# Autodesk Inventor assembly: 基本構造距離センサ2セット配置
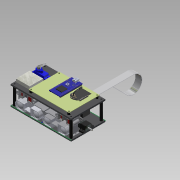
[picture p0: Inventor's stored thumbnail of the model, 180x180]
Saved by Autodesk Inventor 2017 (Build 210142000, 142)
## iProperties
Part Number: 基本構造距離センサ2セット配置
Material: 一般
Document SubType Name: Assembly
Designer: HISAAKI
Author: HISAAKI
## Documents named in this file (19)
- C:\Users\HISAAKI\Documents\LYNCS\CanSat\2017種子島\cansat-structure\基本構造距離センサ2セット配置.iam
- C:\Users\HISAAKI\Documents\LYNCS\CanSat\2017種子島\cansat-structure\既成部品\ブラケット.ipt
- C:\Users\HISAAKI\Documents\LYNCS\CanSat\2017種子島\cansat-structure\既成部品\モータ.ipt
- C:\Users\HISAAKI\Documents\LYNCS\CanSat\2017種子島\cansat-structure\ハブver1.1.ipt
- C:\Users\HISAAKI\Documents\LYNCS\CanSat\2017種子島\cansat-structure\タイヤスポンジ部分.ipt
- C:\Users\HISAAKI\Documents\LYNCS\CanSat\2017種子島\cansat-structure\基本板上.ipt
- C:\Users\HISAAKI\Documents\LYNCS\CanSat\2017種子島\cansat-structure\既成部品\スペーサ.ipt
- C:\Users\HISAAKI\Documents\LYNCS\CanSat\2017種子島\cansat-structure\既成部品\GPSユニット.ipt
- C:\Users\HISAAKI\Documents\LYNCS\CanSat\2017種子島\cansat-structure\基板.ipt
- C:\Users\HISAAKI\Documents\LYNCS\CanSat\2017種子島\cansat-structure\スペーサ5mm.ipt
- C:\Users\HISAAKI\Documents\LYNCS\CanSat\2017種子島\cansat-structure\タイヤプラ板部分.ipt
- C:\Users\HISAAKI\Documents\LYNCS\CanSat\2017種子島\cansat-structure\スタビライザ.ipt
- C:\Users\HISAAKI\Documents\LYNCS\CanSat\2017種子島\cansat-structure\リポ電池黒.ipt
- C:\Users\HISAAKI\Documents\LYNCS\CanSat\2017種子島\cansat-structure\mbed_NXP_LPC1768.ipt
- C:\Users\HISAAKI\Documents\LYNCS\CanSat\2017種子島\cansat-structure\センサ2個積み右.iam
- C:\Users\HISAAKI\Documents\LYNCS\CanSat\2017種子島\cansat-structure\センサ2セット積み左.iam
- C:\Users\HISAAKI\Documents\LYNCS\CanSat\2017種子島\cansat-structure\XBeeProS1.ipt
- C:\Users\HISAAKI\Documents\LYNCS\CanSat\2017種子島\cansat-structure\Tower Pro 9g Micro Servo SG90.ipt
- C:\Users\HISAAKI\Documents\LYNCS\CanSat\2017種子島\cansat-structure\基本板().ipt
## Components (30 placed, 18 different names)
1. モータ:1 — メイト:13, メイト:14, メイト:41, メイト:43, フラッシュ:106
2. モータ:2 — メイト:11, メイト:12, メイト:42, メイト:44, フラッシュ:105
3. ハブver1.1:1 — メイト:11, メイト:12, メイト:17, メイト:18
4. ハブver1.1:2 — メイト:13, メイト:14, メイト:15, メイト:16
5. タイヤスポンジ部分:1 — メイト:15, メイト:16, メイト:62, メイト:63
6. タイヤスポンジ部分:2 — メイト:17, メイト:18, メイト:64, メイト:65
7. 基本板上:1 — メイト:31, メイト:32, フラッシュ:5, メイト:47, メイト:48, メイト:49, メイト:50, メイト:51, メイト:52, メイト:53, メイト:54, メイト:95, メイト:96, メイト:101, メイト:102, メイト:103, メイト:104, メイト:106
8. スペーサ:1 — メイト:99, メイト:102, メイト:103
9. スペーサ:2 — メイト:100, メイト:104, メイト:105, メイト:106, メイト:107
10. スペーサ:3 — メイト:31, メイト:97, メイト:101
11. スペーサ:4
12. GPSユニット:1 — メイト:32, フラッシュ:5
13. ブラケット:1 — メイト:41, メイト:43, メイト:109, メイト:110
14. ブラケット:2 — メイト:42, メイト:44, メイト:93, メイト:111, メイト:112
15. スペーサ5mm:1 — メイト:47, メイト:51, メイト:58
16. スペーサ5mm:2 — メイト:50, メイト:52, メイト:57
17. スペーサ5mm:3 — メイト:48, メイト:54, メイト:55, メイト:59
18. スペーサ5mm:4 — メイト:49, メイト:53, メイト:56
19. 基板:1 — メイト:55, メイト:56, メイト:57, メイト:58, メイト:59, フラッシュ:97, フラッシュ:98, メイト:94, フラッシュ:103, フラッシュ:104
20. タイヤプラ板部分:1 — メイト:62, メイト:63
21. タイヤプラ板部分:2 — メイト:64, メイト:65
22. スタビライザ:1 — メイト:98, メイト:115, メイト:116
23. リポ電池黒:1 — メイト:90, フラッシュ:19, フラッシュ:20
24. リポ電池黒:2 — メイト:90, フラッシュ:19, フラッシュ:20
25. mbed_NXP_LPC1768:1 — フラッシュ:97, フラッシュ:98
26. センサ2個積み右:1 [sub-assembly] — フラッシュ:99, フラッシュ:100, メイト:114
27. センサ2セット積み左:1 [sub-assembly] — フラッシュ:99, フラッシュ:100, メイト:93, メイト:108, メイト:113
28. XBeeProS1:1 — メイト:94, フラッシュ:103, フラッシュ:104
29. Tower Pro 9g Micro Servo SG90:1 — メイト:95, メイト:96
30. 基本板():1 — メイト:97, メイト:98, メイト:99, メイト:100, メイト:105, メイト:107, フラッシュ:105, メイト:108, フラッシュ:106, メイト:109, メイト:110, メイト:111, メイト:112, メイト:113, メイト:114, メイト:115, メイト:116
## Relationships (67: Mate 56, Flush 11)
- メイト:11 [Mate]: モータ:2 ↔ ハブver1.1:1
- メイト:12 [Mate]: モータ:2 ↔ ハブver1.1:1
- メイト:13 [Mate]: モータ:1 ↔ ハブver1.1:2
- メイト:14 [Mate]: モータ:1 ↔ ハブver1.1:2
- メイト:15 [Mate]: ハブver1.1:2 ↔ タイヤスポンジ部分:1
- メイト:16 [Mate]: ハブver1.1:2 ↔ タイヤスポンジ部分:1
- メイト:17 [Mate]: ハブver1.1:1 ↔ タイヤスポンジ部分:2
- メイト:18 [Mate]: ハブver1.1:1 ↔ タイヤスポンジ部分:2
- メイト:31 [Mate]: 基本板上:1 ↔ スペーサ:3
- メイト:32 [Mate]: 基本板上:1 ↔ GPSユニット:1
- フラッシュ:5 [Flush] (10 mm): 基本板上:1 ↔ GPSユニット:1
- メイト:41 [Mate]: モータ:1 ↔ ブラケット:1
- メイト:42 [Mate]: モータ:2 ↔ ブラケット:2
- メイト:43 [Mate]: モータ:1 ↔ ブラケット:1
- メイト:44 [Mate]: モータ:2 ↔ ブラケット:2
- メイト:47 [Mate]: 基本板上:1 ↔ スペーサ5mm:1
- メイト:48 [Mate]: 基本板上:1 ↔ スペーサ5mm:3
- メイト:49 [Mate]: 基本板上:1 ↔ スペーサ5mm:4
- メイト:50 [Mate]: 基本板上:1 ↔ スペーサ5mm:2
- メイト:51 [Mate]: 基本板上:1 ↔ スペーサ5mm:1
- メイト:52 [Mate]: 基本板上:1 ↔ スペーサ5mm:2
- メイト:53 [Mate]: 基本板上:1 ↔ スペーサ5mm:4
- メイト:54 [Mate]: 基本板上:1 ↔ スペーサ5mm:3
- メイト:55 [Mate]: スペーサ5mm:3 ↔ 基板:1
- メイト:56 [Mate]: スペーサ5mm:4 ↔ 基板:1
- メイト:57 [Mate]: スペーサ5mm:2 ↔ 基板:1
- メイト:58 [Mate]: スペーサ5mm:1 ↔ 基板:1
- メイト:59 [Mate]: スペーサ5mm:3 ↔ 基板:1
- メイト:62 [Mate]: タイヤスポンジ部分:1 ↔ タイヤプラ板部分:1
- メイト:63 [Mate]: タイヤスポンジ部分:1 ↔ タイヤプラ板部分:1
- メイト:64 [Mate]: タイヤスポンジ部分:2 ↔ タイヤプラ板部分:2
- メイト:65 [Mate]: タイヤスポンジ部分:2 ↔ タイヤプラ板部分:2
- メイト:90 [Mate]: リポ電池黒:1 ↔ リポ電池黒:2
- フラッシュ:19 [Flush]: リポ電池黒:1 ↔ リポ電池黒:2
- フラッシュ:20 [Flush]: リポ電池黒:1 ↔ リポ電池黒:2
- フラッシュ:97 [Flush]: 基板:1 ↔ mbed_NXP_LPC1768:1
- フラッシュ:98 [Flush] (40 mm): 基板:1 ↔ mbed_NXP_LPC1768:1
- フラッシュ:99 [Flush]: センサ2個積み右:1 ↔ センサ2セット積み左:1
- フラッシュ:100 [Flush]: センサ2個積み右:1 ↔ センサ2セット積み左:1
- メイト:93 [Mate] (3 mm): ブラケット:2 ↔ センサ2セット積み左:1
- メイト:94 [Mate]: 基板:1 ↔ XBeeProS1:1
- フラッシュ:103 [Flush] (10 mm): 基板:1 ↔ XBeeProS1:1
- フラッシュ:104 [Flush] (10 mm): 基板:1 ↔ XBeeProS1:1
- メイト:95 [Mate]: 基本板上:1 ↔ Tower Pro 9g Micro Servo SG90:1
- メイト:96 [Mate]: 基本板上:1 ↔ Tower Pro 9g Micro Servo SG90:1
- メイト:97 [Mate]: スペーサ:3 ↔ 基本板():1
- メイト:98 [Mate]: スタビライザ:1 ↔ 基本板():1
- メイト:99 [Mate]: スペーサ:1 ↔ 基本板():1
- メイト:100 [Mate]: スペーサ:2 ↔ 基本板():1
- メイト:101 [Mate]: 基本板上:1 ↔ スペーサ:3
- メイト:102 [Mate]: 基本板上:1 ↔ スペーサ:1
- メイト:103 [Mate]: 基本板上:1 ↔ スペーサ:1
- メイト:104 [Mate]: 基本板上:1 ↔ スペーサ:2
- メイト:105 [Mate]: スペーサ:2 ↔ 基本板():1
- メイト:106 [Mate]: 基本板上:1 ↔ スペーサ:2
- メイト:107 [Mate]: スペーサ:2 ↔ 基本板():1
- フラッシュ:105 [Flush]: モータ:2 ↔ 基本板():1
- メイト:108 [Mate]: センサ2セット積み左:1 ↔ 基本板():1
- フラッシュ:106 [Flush]: モータ:1 ↔ 基本板():1
- メイト:109 [Mate]: ブラケット:1 ↔ 基本板():1
- メイト:110 [Mate]: ブラケット:1 ↔ 基本板():1
- メイト:111 [Mate]: ブラケット:2 ↔ 基本板():1
- メイト:112 [Mate]: ブラケット:2 ↔ 基本板():1
- メイト:113 [Mate]: センサ2セット積み左:1 ↔ 基本板():1
- メイト:114 [Mate]: センサ2個積み右:1 ↔ 基本板():1
- メイト:115 [Mate]: スタビライザ:1 ↔ 基本板():1
- メイト:116 [Mate]: スタビライザ:1 ↔ 基本板():1
